# Autodesk Inventor assembly: Assembly
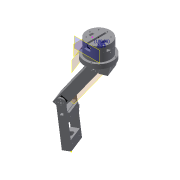
[picture p0: Inventor's stored thumbnail of the model, 180x180]
Saved by Autodesk Inventor 2018 (Build 220112000, 112)
## iProperties
Created: 2017-12-03
Part Number: Assembly
Document SubType Name: Assembly
Designer: Bardo91
Author: Bardo91
## Documents named in this file (14)
- C:\Users\Bardo91\Desktop\hecatonquiros\cad_models\arm_3_dog\serial_model\Assembly.iam
- C:\Users\Bardo91\Desktop\hecatonquiros\cad_models\arm_3_dog\serial_model\arm_0_attachment.ipt
- C:\Users\Bardo91\Desktop\hecatonquiros\cad_models\arm_3_dog\serial_model\arm_0_top.ipt
- C:\Users\Bardo91\Desktop\hecatonquiros\cad_models\arm_3_dog\serial_model\servo_FT_SC.ipt
- C:\Users\Bardo91\Desktop\hecatonquiros\cad_models\arm_3_dog\serial_model\arm_0_bottom.ipt
- C:\Users\Bardo91\Desktop\hecatonquiros\cad_models\arm_3_dog\serial_model\arm_0_bottom_top_lock.ipt
- C:\Users\Bardo91\Desktop\hecatonquiros\cad_models\arm_3_dog\serial_model\servo_FT_SC_horn_1.ipt
- C:\Users\Bardo91\Desktop\hecatonquiros\cad_models\arm_3_dog\serial_model\arm_0_bottom_case.ipt
- C:\Users\Bardo91\Desktop\hecatonquiros\cad_models\arm_3_dog\serial_model\servo_FT_SC_horn_2.ipt
- C:\Users\Bardo91\Desktop\hecatonquiros\cad_models\arm_3_dog\serial_model\arm_1.ipt
- C:\Users\Bardo91\Desktop\hecatonquiros\cad_models\arm_3_dog\serial_model\arm_1_case.ipt
- C:\Users\Bardo91\Desktop\hecatonquiros\cad_models\arm_3_dog\serial_model\arm_2_microservo.ipt
- C:\Users\Bardo91\Desktop\hecatonquiros\cad_models\arm_3_dog\serial_model\arm_2_case_bearing.ipt
- C:\Users\Bardo91\Desktop\hecatonquiros\cad_models\arm_3_dog\serial_model\arm_2_microservo_case.ipt
## Components (17 placed, 13 different names)
1. arm_0_attachment:1 — Mate:1, Mate:2, Mate:3
2. arm_0_top:1 — Mate:1, Mate:2, Mate:3, Mate:4, Mate:5, Mate:6, Mate:7, Flush:1
3. servo_FT_SC:1 — Mate:4, Mate:5, Mate:6, Mate:17, Mate:18
4. servo_FT_SC_horn_1:1 — Mate:17, Mate:18, Mate:19, Mate:20
5. arm_0_bottom:1 — Mate:7, Flush:1, Mate:14, Mate:15, Mate:16, Mate:19, Mate:20, Mate:21, Mate:22, Mate:23, Mate:24, Mate:25, Mate:26, Mate:27
6. arm_0_bottom_top_lock:1 — Mate:14, Mate:15, Mate:16
7. servo_FT_SC:2 — Mate:21, Mate:22, Mate:23, Mate:28, Mate:29, Mate:34
8. arm_0_bottom_case:1 — Mate:24, Mate:25, Mate:26, Mate:27
9. servo_FT_SC_horn_1:2 — Mate:28, Mate:29, Mate:31, Mate:32, Mate:33
10. arm_1:1 — Mate:31, Mate:32, Mate:33, Mate:35, Mate:36, Mate:37, Mate:38, Mate:39, Mate:40, Mate:41, Mate:42
11. servo_FT_SC_horn_2:1 — Mate:34, Mate:35, Mate:36
12. servo_FT_SC:3 — Mate:37, Mate:38, Mate:39, Coincidencia:43, Coincidencia:44, Coincidencia:45
13. arm_1_case:1 — Mate:40, Mate:41, Mate:42
14. arm_2_microservo:1 — Coincidencia:43, Coincidencia:46, Coincidencia:47, Coincidencia:48, Mate:51, Mate:52, Mate:53, Mate:54, Mate:55, Mate:56
15. servo_FT_SC_horn_1:3 — Coincidencia:44, Coincidencia:45, Coincidencia:46, Coincidencia:47, Coincidencia:48
16. arm_2_case_bearing:1 — Mate:51, Mate:52, Mate:53
17. arm_2_microservo_case:1 — Mate:54, Mate:55, Mate:56
## Relationships (48: Mate 47, Flush 1)
- Mate:1: arm_0_attachment:1 ↔ arm_0_top:1
- Mate:2: arm_0_attachment:1 ↔ arm_0_top:1
- Mate:3: arm_0_attachment:1 ↔ arm_0_top:1
- Mate:4: arm_0_top:1 ↔ servo_FT_SC:1
- Mate:5: arm_0_top:1 ↔ servo_FT_SC:1
- Mate:6: arm_0_top:1 ↔ servo_FT_SC:1
- Mate:7: arm_0_top:1 ↔ arm_0_bottom:1
- Flush:1: arm_0_top:1 ↔ arm_0_bottom:1
- Mate:14: arm_0_bottom:1 ↔ arm_0_bottom_top_lock:1
- Mate:15: arm_0_bottom:1 ↔ arm_0_bottom_top_lock:1
- Mate:16: arm_0_bottom:1 ↔ arm_0_bottom_top_lock:1
- Mate:17: servo_FT_SC:1 ↔ servo_FT_SC_horn_1:1
- Mate:18: servo_FT_SC:1 ↔ servo_FT_SC_horn_1:1
- Mate:19: servo_FT_SC_horn_1:1 ↔ arm_0_bottom:1
- Mate:20: servo_FT_SC_horn_1:1 ↔ arm_0_bottom:1
- Mate:21: arm_0_bottom:1 ↔ servo_FT_SC:2
- Mate:22: arm_0_bottom:1 ↔ servo_FT_SC:2
- Mate:23: arm_0_bottom:1 ↔ servo_FT_SC:2
- Mate:24: arm_0_bottom:1 ↔ arm_0_bottom_case:1
- Mate:25: arm_0_bottom:1 ↔ arm_0_bottom_case:1
- Mate:26: arm_0_bottom:1 ↔ arm_0_bottom_case:1
- Mate:27: arm_0_bottom:1 ↔ arm_0_bottom_case:1
- Mate:28: servo_FT_SC:2 ↔ servo_FT_SC_horn_1:2
- Mate:29: servo_FT_SC:2 ↔ servo_FT_SC_horn_1:2
- Mate:31: servo_FT_SC_horn_1:2 ↔ arm_1:1
- Mate:32: servo_FT_SC_horn_1:2 ↔ arm_1:1
- Mate:33: servo_FT_SC_horn_1:2 ↔ arm_1:1
- Mate:34: servo_FT_SC:2 ↔ servo_FT_SC_horn_2:1
- Mate:35: arm_1:1 ↔ servo_FT_SC_horn_2:1
- Mate:36: arm_1:1 ↔ servo_FT_SC_horn_2:1
- Mate:37: arm_1:1 ↔ servo_FT_SC:3
- Mate:38: arm_1:1 ↔ servo_FT_SC:3
- Mate:39: arm_1:1 ↔ servo_FT_SC:3
- Mate:40: arm_1:1 ↔ arm_1_case:1
- Mate:41: arm_1:1 ↔ arm_1_case:1
- Mate:42: arm_1:1 ↔ arm_1_case:1
- Coincidencia:43 [Mate]: servo_FT_SC:3 ↔ arm_2_microservo:1
- Coincidencia:44 [Mate]: servo_FT_SC:3 ↔ servo_FT_SC_horn_1:3
- Coincidencia:45 [Mate]: servo_FT_SC:3 ↔ servo_FT_SC_horn_1:3
- Coincidencia:46 [Mate]: arm_2_microservo:1 ↔ servo_FT_SC_horn_1:3
- Coincidencia:47 [Mate]: arm_2_microservo:1 ↔ servo_FT_SC_horn_1:3
- Coincidencia:48 [Mate]: arm_2_microservo:1 ↔ servo_FT_SC_horn_1:3
- Mate:51: arm_2_microservo:1 ↔ arm_2_case_bearing:1
- Mate:52: arm_2_microservo:1 ↔ arm_2_case_bearing:1
- Mate:53: arm_2_microservo:1 ↔ arm_2_case_bearing:1
- Mate:54: arm_2_microservo:1 ↔ arm_2_microservo_case:1
- Mate:55: arm_2_microservo:1 ↔ arm_2_microservo_case:1
- Mate:56: arm_2_microservo:1 ↔ arm_2_microservo_case:1
